# Autodesk Inventor assembly: Solenoid
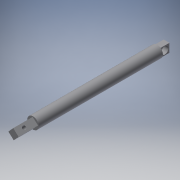
[picture p0: Inventor's stored thumbnail of the model, 180x180]
Saved by Autodesk Inventor 2018 (Build 220112000, 112)
## iProperties
Created: 2018-05-31
Part Number: Solenoid
Document SubType Name: Assembly
Designer: choices
Author: choices
## Documents named in this file (3)
- C:\Users\choices\Documents\Solenoid.iam
- C:\Users\choices\Documents\SolenoidArm.ipt
- C:\Users\choices\Documents\SolenoidCase.ipt
## Components (2 placed, 2 different names)
1. SolenoidArm:1 — Mate:1, Mate:2
2. SolenoidCase:1 — Mate:1, Mate:2
## Relationships (2: Mate 2)
- Mate:1: SolenoidArm:1 ↔ SolenoidCase:1
- Mate:2: SolenoidArm:1 ↔ SolenoidCase:1
